# Autodesk Inventor assembly: Shock Absorber
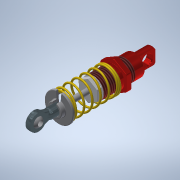
[picture p0: Inventor's stored thumbnail of the model, 180x180]
Saved by Autodesk Inventor 2022.3 (Build 263350000, 350)
## iProperties
Created: 2019-12-02
Part Number: Shock Absorber
Document SubType Name: Assembly
Designer: Jopa
Author: Jopa
## Documents named in this file (5)
- D:\Luis\Desktop\ESPOL\9 semestre\Itinerario\PIEZAS\PX9200-18_Front-Rear_Shock_Absorber\PX9200-18_Front-Rear_Shock_Absorber.iam
- D:\Luis\Desktop\ESPOL\9 semestre\Itinerario\PIEZAS\PX9200-18_Front-Rear_Shock_Absorber\Shock Spring Adjustment Nut.ipt
- D:\Luis\Desktop\ESPOL\9 semestre\Itinerario\PIEZAS\PX9200-18_Front-Rear_Shock_Absorber\Suspension Spring.ipt
- D:\Luis\Desktop\ESPOL\9 semestre\Itinerario\PIEZAS\PX9200-18_Front-Rear_Shock_Absorber\Shock Body\Shock Body.iam
- D:\Luis\Desktop\ESPOL\9 semestre\Itinerario\PIEZAS\PX9200-18_Front-Rear_Shock_Absorber\Shock Strut\Shock Strut.iam
## Components (4 placed, 4 different names)
1. Shock Spring Adjustment Nut:1 — Mate:1, Mate:2, Flush:1, Angle:1, Mate MID
2. Suspension Spring:1 — Mate:1, Mate:4, Mate MID
3. Shock Body:1 [sub-assembly] — Mate:2, Flush:1, Angle:1, Mate:3, Angle:2, Mate OPEN, Mate CLOSE
4. Shock Strut:1 [sub-assembly] — Mate:3, Mate:4, Angle:2, Mate OPEN, Mate CLOSE
## Relationships (10: Mate 7, Angle 2, Flush 1)
- Mate:1: Shock Spring Adjustment Nut:1 ↔ Suspension Spring:1
- Mate:2: Shock Spring Adjustment Nut:1 ↔ Shock Body:1
- Flush:1 (-10.1676 mm): Shock Spring Adjustment Nut:1 ↔ Shock Body:1
- Angle:1 (0 deg): Shock Spring Adjustment Nut:1 ↔ Shock Body:1
- Mate:3: Shock Body:1 ↔ Shock Strut:1
- Mate:4: Suspension Spring:1 ↔ Shock Strut:1
- Angle:2 (0 deg): Shock Body:1 ↔ Shock Strut:1
- Mate OPEN: Shock Body:1 ↔ Shock Strut:1
- Mate CLOSE: Shock Body:1 ↔ Shock Strut:1
- Mate MID: Shock Spring Adjustment Nut:1 ↔ Suspension Spring:1
